# Autodesk Inventor assembly: servo-dummy
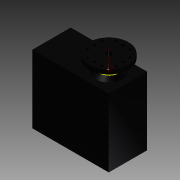
[picture p0: Inventor's stored thumbnail of the model, 180x180]
Saved by Autodesk Inventor 2013 (Build 170138000, 138)
## iProperties
Created: 2013-09-15
Part Number: servo-dummy
Document SubType Name: Assembly
Designer: Ian
Mass: 34.6585 g
Surface Area: 81.8776 cm^2
Volume: 32.6967 cm^3
Density: 1.06 g/cm^3
Author: Ian
## Documents named in this file (3)
- C:\Users\Ian\Documents\Inventor\xyPartStorage\servo-dummy\servo-dummy.iam
- C:\Users\Ian\Documents\Inventor\xyPartStorage\servo-dummy\body.ipt
- C:\Users\Ian\Documents\Inventor\xyPartStorage\servo-dummy\horn01.ipt
## Components (2 placed, 2 different names)
1. body:1 — Insert:1
2. horn01:1 — Insert:1
## Relationships (1: Insert 1)
- Insert:1 (-6.35 mm): body:1 ↔ horn01:1
